# Autodesk Inventor assembly: ViaductPillar_SingleSpan-05us
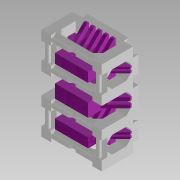
[picture p0: Inventor's stored thumbnail of the model, 180x180]
Saved by Autodesk Inventor 2021 (Build 250183000, 183)
## iProperties
Created: 2021-03-15
Part Number: ViaductPillar_SingleSpan-05us
Document SubType Name: Assembly
Designer: kumagai
Author: kumagai
## Documents named in this file (12)
- X:\Develop\CAD\PlaRails\ViaductPillarUnit\ViaductPillar_SingleSpan_Doublelane.iam
- X:\Develop\CAD\PlaRails\ViaductPillarUnit\VPU_EdgeBottom.ipt
- X:\Develop\CAD\PlaRails\ViaductPillarUnit\VPU_EdgeTop.ipt
- X:\Develop\CAD\PlaRails\GlobalParameter.ipt
- X:\Develop\CAD\PlaRails\ViaductPillarUnit\VPU_SupportSingle.ipt
- X:\Develop\CAD\PlaRails\ViaductPillarUnit\VPU_IC_Bottom.ipt
- X:\Develop\CAD\PlaRails\ViaductPillarUnit\VPU_IC_Top.ipt
- X:\Develop\CAD\PlaRails\ViaductPillarUnit\VPU_IC_SupportSingle.ipt
- ViaductPillar_SingleSpan-05u.iam
- ViaductPillar_SingleSpan-05us.iam
- ViaductPillar_SingleSpan-1u.iam
- ViaductPillar_SingleSpan-1us.iam
## Components (15 placed, 6 different names)
1. VPU_IC_Bottom:1 — フラッシュ:16, フラッシュ:18, フラッシュ:20
2. VPU_IC_Bottom:2 — フラッシュ:17, フラッシュ:19, フラッシュ:21
3. VPU_IC_Top:1 — フラッシュ:11, フラッシュ:13, フラッシュ:14, フラッシュ:22
4. VPU_IC_Top:2 — フラッシュ:10, フラッシュ:12, フラッシュ:15
5. VPU_IC_SupportSingle:1 — フラッシュ:22, フラッシュ:23, フラッシュ:24
6. VPU_SupportSingle:1 — フラッシュ:7, フラッシュ:8, フラッシュ:9, フラッシュ:23, フラッシュ:24
7. VPU_EdgeTop:2 — メイト:2, フラッシュ:5, フラッシュ:6, フラッシュ:11, フラッシュ:13, フラッシュ:14
8. VPU_EdgeTop:1 — フラッシュ:3, フラッシュ:4, メイト:2, フラッシュ:5, フラッシュ:6, メイト:3, フラッシュ:10, フラッシュ:12, フラッシュ:15
9. VPU_EdgeBottom:2 — メイト:1, フラッシュ:1, フラッシュ:2, フラッシュ:16, フラッシュ:18, フラッシュ:20
10. VPU_EdgeBottom:1 — メイト:1, フラッシュ:1, フラッシュ:2, フラッシュ:3, フラッシュ:4, メイト:3, フラッシュ:17, フラッシュ:19, フラッシュ:21
11. VPU_SupportSingle:2
12. VPU_EdgeTop:3
13. VPU_EdgeTop:4
14. VPU_EdgeBottom:3
15. VPU_EdgeBottom:4
## Component patterns: (2 elements, first: VPU_SupportSingle:1 + VPU_EdgeTop:2 + VPU_EdgeTop:1 + VPU_EdgeBottom:2 + VPU_EdgeBottom:1)
## Relationships (27: Flush 24, Mate 3)
- メイト:1 [Mate]: VPU_EdgeBottom:2 ↔ VPU_EdgeBottom:1
- フラッシュ:1 [Flush]: VPU_EdgeBottom:2 ↔ VPU_EdgeBottom:1
- フラッシュ:2 [Flush]: VPU_EdgeBottom:2 ↔ VPU_EdgeBottom:1
- フラッシュ:3 [Flush]: VPU_EdgeTop:1 ↔ VPU_EdgeBottom:1
- フラッシュ:4 [Flush]: VPU_EdgeTop:1 ↔ VPU_EdgeBottom:1
- メイト:2 [Mate]: VPU_EdgeTop:2 ↔ VPU_EdgeTop:1
- フラッシュ:5 [Flush]: VPU_EdgeTop:2 ↔ VPU_EdgeTop:1
- フラッシュ:6 [Flush]: VPU_EdgeTop:2 ↔ VPU_EdgeTop:1
- メイト:3 [Mate] (-33 mm): VPU_EdgeTop:1 ↔ VPU_EdgeBottom:1
- フラッシュ:7 [Flush]: VPU_SupportSingle:1
- フラッシュ:8 [Flush]: VPU_SupportSingle:1
- フラッシュ:9 [Flush]: VPU_SupportSingle:1
- フラッシュ:10 [Flush]: VPU_IC_Top:2 ↔ VPU_EdgeTop:1
- フラッシュ:11 [Flush]: VPU_IC_Top:1 ↔ VPU_EdgeTop:2
- フラッシュ:12 [Flush]: VPU_IC_Top:2 ↔ VPU_EdgeTop:1
- フラッシュ:13 [Flush]: VPU_IC_Top:1 ↔ VPU_EdgeTop:2
- フラッシュ:14 [Flush]: VPU_IC_Top:1 ↔ VPU_EdgeTop:2
- フラッシュ:15 [Flush]: VPU_IC_Top:2 ↔ VPU_EdgeTop:1
- フラッシュ:16 [Flush]: VPU_IC_Bottom:1 ↔ VPU_EdgeBottom:2
- フラッシュ:17 [Flush]: VPU_IC_Bottom:2 ↔ VPU_EdgeBottom:1
- フラッシュ:18 [Flush]: VPU_IC_Bottom:1 ↔ VPU_EdgeBottom:2
- フラッシュ:19 [Flush]: VPU_IC_Bottom:2 ↔ VPU_EdgeBottom:1
- フラッシュ:20 [Flush]: VPU_IC_Bottom:1 ↔ VPU_EdgeBottom:2
- フラッシュ:21 [Flush]: VPU_IC_Bottom:2 ↔ VPU_EdgeBottom:1
- フラッシュ:22 [Flush]: VPU_IC_Top:1 ↔ VPU_IC_SupportSingle:1
- フラッシュ:23 [Flush]: VPU_IC_SupportSingle:1 ↔ VPU_SupportSingle:1
- フラッシュ:24 [Flush]: VPU_IC_SupportSingle:1 ↔ VPU_SupportSingle:1
## Named parameters: ViaductHeight = 66 mm, HeightRatio = 0.5, FaceShift = 0 mm, DoubleWidth = 60 mm
